# Autodesk Inventor assembly: 2018ToughboxMicrowithAngledPlateAndCim
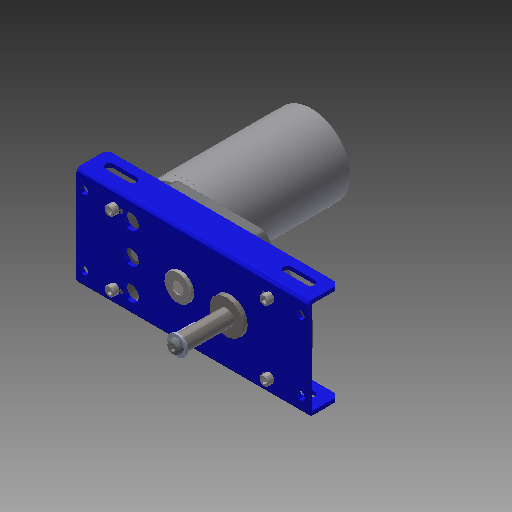
[picture p0: Inventor's stored thumbnail of the model, 512x512]
Saved by Autodesk Inventor 2018 (Build 220112000, 112)
## iProperties
Created: 2015-11-11
Part Number: 2018ToughboxMicrowithAngledPlateAndCim
Description: STEP AP214
Document SubType Name: Assembly
Designer: Apple
Sending System: SolidWorks 2014
Preprocessor: SwSTEP 2.0
Title: am-3231 Toughbox Micro with Angled Plate.STEP
Revision Number: ANY
## Documents named in this file (4)
- C:\Users\Apple\Documents\Inventor\2018 PowerUp\2018ToughboxMicrowithAngledPlateAndCim.iam
- C:\Users\Apple\Documents\Inventor\2018 PowerUp\AndyMark\Sheet Metal Front Plate Rev 7.ipt
- C:\Users\Apple\Documents\Inventor\2018 PowerUp\AndyMark\Molded Assembly Rev 7 with am-0153 shaft_Long Micro Shaft.iam
- C:\Users\Apple\Documents\Inventor\2018 PowerUp\CIM motor-1.ipt
## Components (3 placed, 3 different names)
1. Sheet Metal Front Plate Rev 7_1
2. Molded Assembly Rev 7 with am-0153 shaft_Long Micro Shaft_2 [sub-assembly] — Mate:1, Mate:2
3. CIM motor-1:1 — Mate:1, Mate:2
## Relationships (2: Mate 2)
- Mate:1: Molded Assembly Rev 7 with am-0153 shaft_Long Micro Shaft_2 ↔ CIM motor-1:1
- Mate:2: Molded Assembly Rev 7 with am-0153 shaft_Long Micro Shaft_2 ↔ CIM motor-1:1
